# Autodesk Inventor assembly: FrameV2
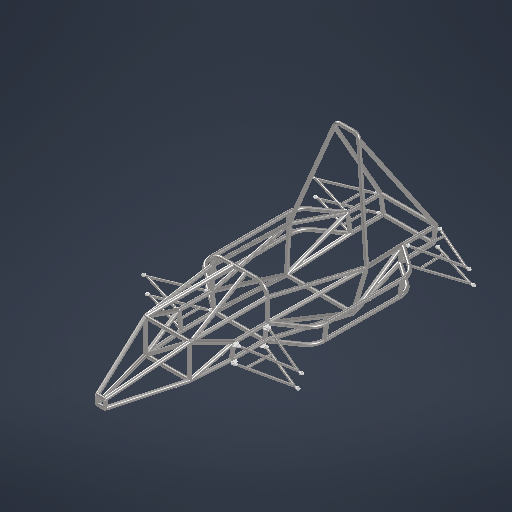
[picture p0: Inventor's stored thumbnail of the model, 512x512]
Saved by Autodesk Inventor 2026.1 (Build 301233000, 233)
## iProperties
Created: 2026-06-05
Part Number: FrameV2
Document SubType Name: Assembly
Designer: tasle
_SolveAssemblyDoc: Frame Generator Solve Assembly
_Version: 15.0.0
Author: tasle
## Documents named in this file (5)
- C:\Users\share\OneDrive\Documents\Personal Projects\GOGO Kart\CAD\GOGO_KART_FSAE\Frame + Suspension CAD\FrameV2 - Copy.iam
- C:\Users\share\OneDrive\Documents\Personal Projects\GOGO Kart\CAD\GOGO_KART_FSAE\PrelimFrame.ipt
- C:\Users\share\OneDrive\Documents\Personal Projects\GOGO Kart\CAD\GOGO_KART_FSAE\FrameV2\Frame\Frame 1780692296746.iam
- C:\Users\share\OneDrive\Documents\Personal Projects\GOGO Kart\CAD\GOGO_KART_FSAE\Shareef\Suspension Parts\Front Upper Arm\Front_Upper_Arm_Assembly.iam
- C:\Users\share\OneDrive\Documents\Personal Projects\GOGO Kart\CAD\GOGO_KART_FSAE\Shareef\Suspension Parts\Front Upper Arm\Rod End Bracket.ipt
## Components (14 placed, 4 different names)
1. PrelimFrame:1 — Flush:1, Mate:5
2. Frame 1780692296746:1 [sub-assembly]
3. Front_Upper_Arm_Assembly:1 [sub-assembly]
4. Rod End Bracket:1 — Mate:1, Insert:1
5. Rod End Bracket:2 — Mate:3
6. Rod End Bracket:3 — Mate:2
7. Rod End Bracket:4 — Mate:4
8. Front_Upper_Arm_Assembly:2 [sub-assembly]
9. Front_Upper_Arm_Assembly:3 [sub-assembly] — Insert:1
10. Front_Upper_Arm_Assembly:4 [sub-assembly]
11. Front_Upper_Arm_Assembly:5 [sub-assembly]
12. Front_Upper_Arm_Assembly:6 [sub-assembly]
13. Front_Upper_Arm_Assembly:7 [sub-assembly]
14. Front_Upper_Arm_Assembly:8 [sub-assembly]
## Relationships (8: Mate 5, Flush 1, Angle 1, Insert 1)
- Flush:1 (17.78 mm): PrelimFrame:1
- Mate:1: Rod End Bracket:1
- Mate:2: Rod End Bracket:3
- Mate:3: Rod End Bracket:2
- Mate:4: Rod End Bracket:4
- Mate:5: PrelimFrame:1
- Angle:1 (90 deg)
- Insert:1: Rod End Bracket:1 ↔ Front_Upper_Arm_Assembly:3
